# Autodesk Inventor assembly: subsystem_1
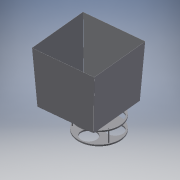
[picture p0: Inventor's stored thumbnail of the model, 180x180]
Saved by Autodesk Inventor 2019 (Build 230136000, 136)
## iProperties
Created: 2020-02-29
Part Number: subsystem_1
Document SubType Name: Assembly
Designer: Jayadev
Author: Jayadev
## Documents named in this file (6)
- G:\Inventor 2019\subsystem_1.iam
- G:\Inventor 2019\subsystem_1_basket.ipt
- G:\Inventor 2019\subsystem_1_feeder_disk.iam
- G:\Inventor 2019\subsystem_1_bsket_feeder_pipe.ipt
- G:\Inventor 2019\subsystem_1_feeder_basket_rod.ipt
- G:\Inventor 2019\subsystem_1_basket_support_rod.ipt
## Components (5 placed, 5 different names)
1. subsystem_1_basket:1 — Mate:1, Flush:1, Mate:4, Flush:3, Mate:6, Flush:5
2. subsystem_1_feeder_disk:1 [sub-assembly] — Mate:2, Flush:2, Mate:3
3. subsystem_1_bsket_feeder_pipe:1 — Mate:1, Flush:1
4. subsystem_1_feeder_basket_rod:1 — Mate:2, Flush:2, Mate:3, Mate:4, Flush:3
5. subsystem_1_basket_support_rod:1 — Mate:6, Flush:5
## Relationships (9: Mate 5, Flush 4)
- Mate:1: subsystem_1_basket:1 ↔ subsystem_1_bsket_feeder_pipe:1
- Flush:1: subsystem_1_basket:1 ↔ subsystem_1_bsket_feeder_pipe:1
- Mate:2: subsystem_1_feeder_disk:1 ↔ subsystem_1_feeder_basket_rod:1
- Flush:2: subsystem_1_feeder_disk:1 ↔ subsystem_1_feeder_basket_rod:1
- Mate:3: subsystem_1_feeder_disk:1 ↔ subsystem_1_feeder_basket_rod:1
- Mate:4: subsystem_1_basket:1 ↔ subsystem_1_feeder_basket_rod:1
- Flush:3: subsystem_1_basket:1 ↔ subsystem_1_feeder_basket_rod:1
- Mate:6: subsystem_1_basket:1 ↔ subsystem_1_basket_support_rod:1
- Flush:5: subsystem_1_basket:1 ↔ subsystem_1_basket_support_rod:1
